# Autodesk Inventor assembly: SCSTR6-8
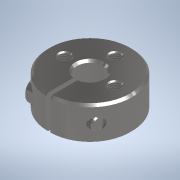
[picture p0: Inventor's stored thumbnail of the model, 180x180]
Saved by Autodesk Inventor 2022 (Build 260153000, 153)
## iProperties
Category: PARTsolutions
Company: MISUMI
Part Number: SCSTR6-8
Catalog Web Link: www.cadenas.de
Description: SCST, PSCST, SSCST, SCSTR, PSCSTR, SSCSTR-Shaft Collars - 3 Holes/3 Taps
Vendor: MISUMI
Document SubType Name: Assembly
Designer: partserver
Manufacturer: MISUMI
Mass: 2.06771 g
Surface Area: 17.5201 cm^2
Volume: 2.06771 cm^3
Density: 1 g/cm^3
PSOL_IDENT_0: {$CADENAS_DATA\23d-libs\misumi\metric\03_set_collars\scst_asmtab.prj},220 {VTYP=3D},{STYP=ASSTAB},{N
PSOL_IDENT_1: B=SCSTR6-8},{LINA=SCSTR6-8},{NN=SCST, PSCST, SSCST, SCSTR, PSCSTR, SSCSTR},{DATE=30.06.2021 12:52:05
PSOL_IDENT_2: },{GEOMDATE=30.10.2015 01:45:58},{VERSION=},{LINEID=220},{WBVAR=TS,MAT,ST,BS},{WBNUMERIC=BS}  {NB=SC
PSOL_IDENT_3: STR6-8},{LINA=SCSTR6-8},{KT=DUMMY},{PN=SCSTR6-8},{TYPE=SCSTR},{TS=3T},{TSALG= '3H' , '3-Hole' , '3T'
PSOL_IDENT_4: , '3-Tapped' },{MAT=S45C},{ST=BO},{STALG= 'BO' , 'Black Oxide' , 'ENP' , 'Electroless Nickel Platin
PSOL_IDENT_5: g' },{AC=Hex Socket Head Cap Screw 1 pc.},{ACMAT=4137 Alloy Steel},{D=6},{BS=8},{BALG= 8 , 10 },{D1=
PSOL_IDENT_6: 20},{M=M3},{M3D=3},{DD=3.4},{R=3.00},{W=1.0},{X=6.0},{Y=4},{P=12},{C=0.5},{S=0.0},{M1=M3},{M13D=3},{
PSOL_IDENT_7: L=12},{PPATH=scst/scst_templ.prj}
NB: SCSTR6-8
NN: SCST, PSCST, SSCST, SCSTR, PSCSTR, SSCSTR
NT: Shaft Collars - 3 Holes/3 Taps
NBSYN: $PN.
LINA: SCSTR6-8
CATALOG: Misumi
PN: SCSTR6-8
TS: 3-Tapped
MAT: 1045 Carbon Steel
ST: Black Oxide
AC: Hex Socket Head Cap Screw 1 pc.
ACMAT: 4137 Alloy Steel
D: 6
BS: 8
D1: 20
M: M3
DD: 3.4
R: 3
W: 1
X: 6
Y: 4
P: 12
C: 0.5
S: 0
M1: M3
SUPPLIER: MISUMI
ARTICLENO: SCSTR6-8
BOMINFO: SCSTR6-8
CREATOR: CADENAS GmbH
Title: SCSTR6-8
Author: Cadenas PARTsolutions
Comments: Shaft Collars - 3 Holes/3 Taps
## Documents named in this file (3)
- C:\Users\yuto6\Box\Public_Share\キャチロボバトルコンテスト2021\CAD\catchrobo_hardware\assy-shooter\SCSTR6-8.iam
- C:\Users\yuto6\Box\Public_Share\キャチロボバトルコンテスト2021\CAD\catchrobo_hardware\assy-shooter\SCSTR6-8b.ipt
- C:\Users\yuto6\Box\Public_Share\キャチロボバトルコンテスト2021\CAD\catchrobo_hardware\assy-shooter\BOLT3-12.ipt
## Components (2 placed, 2 different names)
1. SCSTR6-8b:1 — to_bolt_XY@1 <-> to_cp_XY@2, to_bolt_Z@1 <-> to_cp_Z@2, to_bolt_YZ@1 <-> to_cp_YZ@2
2. BOLT3-12:1 — to_bolt_XY@1 <-> to_cp_XY@2, to_bolt_Z@1 <-> to_cp_Z@2, to_bolt_YZ@1 <-> to_cp_YZ@2
## Relationships (3: Mate 2, Angle 1)
- to_bolt_XY@1 <-> to_cp_XY@2 [Mate]: SCSTR6-8b:1 ↔ BOLT3-12:1
- to_bolt_Z@1 <-> to_cp_Z@2 [Mate]: SCSTR6-8b:1 ↔ BOLT3-12:1
- to_bolt_YZ@1 <-> to_cp_YZ@2 [Angle] (0 deg): SCSTR6-8b:1 ↔ BOLT3-12:1
